# Autodesk Inventor assembly: RearAxle
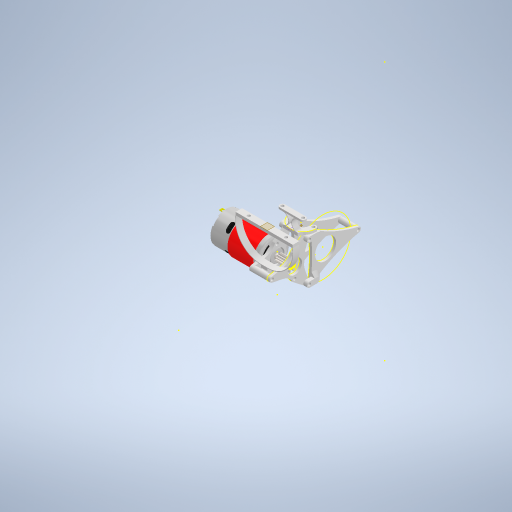
[picture p0: Inventor's stored thumbnail of the model, 512x512]
Saved by Autodesk Inventor 2024 (Build 280153020, 153B)
## iProperties
Created: 2024-04-17
Part Number: RearAxle
Document SubType Name: Assembly
Designer: lvrectanus0
Author: lvrectanus0
## Documents named in this file (9)
- C:\Users\lvrectanus0\Documents\Github\SPARKLabs-ArduinoProjects\project\CAD\RearAxle.iam
- C:\Users\lvrectanus0\Documents\Github\SPARKLabs-ArduinoProjects\project\CAD\am-3775a_12T 775 RedLine with 12T Pinion.iam
- C:\Users\lvrectanus0\Documents\Github\SPARKLabs-ArduinoProjects\project\CAD\MotorHolder.ipt
- C:\Users\lvrectanus0\Documents\Github\SPARKLabs-ArduinoProjects\project\CAD\AxleMount.ipt
- C:\Users\lvrectanus0\Documents\Github\SPARKLabs-ArduinoProjects\project\CAD\MotorMountSpacerConnector.ipt
- C:\Users\lvrectanus0\Documents\Github\SPARKLabs-ArduinoProjects\project\CAD\AxleMount_MIR.ipt
- C:\Users\lvrectanus0\Documents\Github\SPARKLabs-ArduinoProjects\project\CAD\MototMountSpacer.ipt
- C:\Users\lvrectanus0\Documents\Github\SPARKLabs-ArduinoProjects\project\CAD\MotorMountTopSuspension.ipt
- C:\Users\lvrectanus0\Documents\Github\SPARKLabs-ArduinoProjects\project\CAD\MotorMountBackSuspension.ipt
## Components (9 placed, 8 different names)
1. am-3775a_12T 775 RedLine with 12T Pinion:1 [sub-assembly] — Flush:1
2. MotorHolder:1 — Flush:1, Flush:3, Flush:4, Mate:2
3. AxleMount:1 — Flush:3, Flush:5, Mate:9, Mate:11, Angle:1
4. MotorMountSpacerConnector:1 — Flush:4, Mate:1, Mate:3, Flush:7
5. MotorHolder:2 — Mate:1, Mate:2, Mate:3, Mate:4, Mate:5, Mate:6
6. AxleMount_MIR:1 — Mate:4, Mate:5, Mate:6, Mate:10, Mate:12
7. MototMountSpacer:1 — Flush:5
8. MotorMountTopSuspension:1 — Flush:6, Mate:16
9. MotorMountBackSuspension:1 — Flush:7, Mate:16
## Relationships (21: Mate 14, Flush 6, Angle 1)
- Flush:1: am-3775a_12T 775 RedLine with 12T Pinion:1 ↔ MotorHolder:1
- Flush:3: MotorHolder:1 ↔ AxleMount:1
- Flush:4: MotorHolder:1 ↔ MotorMountSpacerConnector:1
- Mate:1: MotorMountSpacerConnector:1 ↔ MotorHolder:2
- Mate:2: MotorHolder:1 ↔ MotorHolder:2
- Mate:3: MotorMountSpacerConnector:1 ↔ MotorHolder:2
- Mate:4: MotorHolder:2 ↔ AxleMount_MIR:1
- Mate:5: MotorHolder:2 ↔ AxleMount_MIR:1
- Mate:6: MotorHolder:2 ↔ AxleMount_MIR:1
- Flush:5: AxleMount:1 ↔ MototMountSpacer:1
- Mate:9: AxleMount:1
- Mate:10: AxleMount_MIR:1
- Mate:11: AxleMount:1
- Mate:12: AxleMount_MIR:1
- Mate:13
- Mate:14
- Mate:15
- Angle:1 (0 deg): AxleMount:1
- Flush:6: MotorMountTopSuspension:1
- Flush:7: MotorMountSpacerConnector:1 ↔ MotorMountBackSuspension:1
- Mate:16: MotorMountTopSuspension:1 ↔ MotorMountBackSuspension:1
